# Autodesk Inventor assembly: Nathan_RobotArm_Assembly
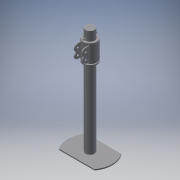
[picture p0: Inventor's stored thumbnail of the model, 180x180]
Saved by Autodesk Inventor 2016 (Build 200138000, 138)
## iProperties
Created: 2017-03-30
Part Number: Nathan_RobotArm_Assembly
Document SubType Name: Assembly
Designer: brandn
Author: brandn
## Documents named in this file (7)
- \\mps\fs\StudentHome\Student2019\brandn\My Documents\Nathan CAD\Nathan_RobotArm_Assembly.iam
- \\mps\fs\StudentHome\Student2019\brandn\My Documents\Nathan CAD\Nathan_RobotArm_Shaft.ipt
- \\mps\fs\StudentHome\Student2019\brandn\My Documents\Nathan CAD\Nathan_RobotArm_TwistPart.ipt
- \\mps\fs\StudentHome\Student2019\brandn\My Documents\Nathan CAD\Nathan_RobotArm_Washer.ipt
- \\mps\fs\StudentHome\Student2019\brandn\My Documents\Nathan CAD\Nathan_RobotArm_B.ipt
- \\mps\fs\StudentHome\Student2019\brandn\My Documents\Nathan CAD\Nathan_RobotArm_Stopper.ipt
- \\mps\fs\StudentHome\Student2019\brandn\My Documents\Nathan CAD\Nathan_RobotArm_Base.ipt
## Components (7 placed, 6 different names)
1. Nathan_RobotArm_Shaft:1 — Rotational:1, Rigid:1, Rigid:4, Rigid:5
2. Nathan_RobotArm_TwistPart:1 — Rotational:1, Rigid:2, Rigid:3
3. Nathan_RobotArm_Washer:1 — Rigid:1
4. Nathan_RobotArm_B:1 — Rigid:2
5. Nathan_RobotArm_B:2 — Rigid:3
6. Nathan_RobotArm_Stopper:1 — Rigid:4
7. Nathan_RobotArm_Base:1 — Rigid:5
## Relationships (6: WeldJoint 5, RevoluteJoint 1)
- Rotational:1 [RevoluteJoint] (-101.6 mm): Nathan_RobotArm_Shaft:1 ↔ Nathan_RobotArm_TwistPart:1
- Rigid:1 [WeldJoint] (-73.66 mm): Nathan_RobotArm_Shaft:1 ↔ Nathan_RobotArm_Washer:1
- Rigid:2 [WeldJoint]: Nathan_RobotArm_TwistPart:1 ↔ Nathan_RobotArm_B:1
- Rigid:3 [WeldJoint]: Nathan_RobotArm_TwistPart:1 ↔ Nathan_RobotArm_B:2
- Rigid:4 [WeldJoint]: Nathan_RobotArm_Shaft:1 ↔ Nathan_RobotArm_Stopper:1
- Rigid:5 [WeldJoint]: Nathan_RobotArm_Shaft:1 ↔ Nathan_RobotArm_Base:1
